# Autodesk Inventor assembly: Hopper_And_Connecting_Plate
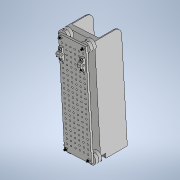
[picture p0: Inventor's stored thumbnail of the model, 180x180]
Saved by Autodesk Inventor 2022 (Build 260153000, 153)
## iProperties
Created: 2022-01-17
Part Number: Hopper_And_Connecting_Plate
Document SubType Name: Assembly
Designer: Work
Author: Work
## Documents named in this file (3)
- C:\Users\Work\Desktop\NewHopper\Hopper_And_Connecting_Plate.iam
- C:\Users\Work\Desktop\NewHopper\Recycling_Hopper.iam
- C:\Users\Work\Desktop\DSW\Wk-1\_Resources\Project 3 Autodesk Inventor Files\2. Hopper Assembly\Connecting_Plate.iam
## Components (2 placed, 2 different names)
1. Recycling_Hopper:1 [sub-assembly] — Mate:1, Mate:2, Mate:3, Mate:4
2. Connecting_Plate:1 [sub-assembly] — Mate:1, Mate:2, Mate:3, Mate:4
## Relationships (4: Mate 4)
- Mate:1: Recycling_Hopper:1 ↔ Connecting_Plate:1
- Mate:2: Recycling_Hopper:1 ↔ Connecting_Plate:1
- Mate:3: Recycling_Hopper:1 ↔ Connecting_Plate:1
- Mate:4: Recycling_Hopper:1 ↔ Connecting_Plate:1
